# Autodesk Inventor assembly: Geeetech GT9S2 Extruder
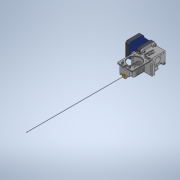
[picture p0: Inventor's stored thumbnail of the model, 180x180]
Saved by Autodesk Inventor 2020 (Build 240168000, 168)
## iProperties
Created: 2018-11-15
Part Number: Geeetech GT9S2 Extruder
Document SubType Name: Assembly
Designer: LillaHunden
Mass: 246.363 g
Surface Area: 552.129 cm^2
Volume: 126.998 cm^3
Density: 1.9399 g/cm^3
Author: LillaHunden
## Documents named in this file (24)
- C:\Users\LillaHunden\Documents\Inventor\3dprinter\3dPrinter\Geeetech GT9S2 Extruder\Geeetech GT9S2 Extruder.iam
- C:\Users\LillaHunden\Documents\Inventor\3dprinter\3dPrinter\Geeetech GT9S2 Extruder\Cooling fin.ipt
- C:\Users\LillaHunden\Documents\Inventor\3dprinter\3dPrinter\Geeetech GT9S2 Extruder\extruder body.ipt
- C:\Users\LillaHunden\Documents\Inventor\3dprinter\3dPrinter\Geeetech GT9S2 Extruder\fan bracket.ipt
- C:\Users\LillaHunden\Documents\Inventor\3dprinter\3dPrinter\Geeetech GT9S2 Extruder\feeder tube.ipt
- C:\Users\LillaHunden\Documents\Inventor\3dprinter\3dPrinter\Geeetech GT9S2 Extruder\hotend.ipt
- C:\Users\LillaHunden\Documents\Inventor\3dprinter\3dPrinter\Geeetech GT9S2 Extruder\nozzel.ipt
- C:\Users\LillaHunden\Documents\Inventor\3dprinter\3dPrinter\Geeetech GT9S2 Extruder\Geeetech GT9S2 Extruder\Design Accelerator\Bolted Connection1.iam
- C:\Users\LillaHunden\Documents\Inventor\3dprinter\3dPrinter\Geeetech GT9S2 Extruder\Geeetech GT9S2 Extruder\Design Accelerator\Bolted Connection2.iam
- C:\Users\LillaHunden\Documents\Inventor\3dprinter\3dPrinter\Geeetech GT9S2 Extruder\roller bracket.ipt
- C:\Users\LillaHunden\Documents\Inventor\3dprinter\3dPrinter\Geeetech GT9S2 Extruder\roller bearing.ipt
- C:\Users\LillaHunden\Documents\Inventor\3dprinter\3dPrinter\Geeetech GT9S2 Extruder\roller pin.ipt
- C:\Users\LillaHunden\Documents\Inventor\3dprinter\3dPrinter\Geeetech GT9S2 Extruder\roller.ipt
- C:\Users\LillaHunden\Documents\Inventor\3dprinter\3dPrinter\Nema17 import\Nema 17HS4401-S.ipt
- C:\Users\LillaHunden\Documents\Inventor\3dprinter\3dPrinter\Geeetech GT9S2 Extruder\Geeetech GT9S2 Extruder\Design Accelerator\Bolted Connection3.iam
- C:\Users\LillaHunden\Documents\Inventor\3dprinter\3dPrinter\Geeetech GT9S2 Extruder\Fillament hob.ipt
- C:\Users\LillaHunden\Documents\Inventor\3dprinter\3dPrinter\Geeetech GT9S2 Extruder\fillament guide screw.ipt
- C:\Users\LillaHunden\Documents\Inventor\3dprinter\3dPrinter\Geeetech GT9S2 Extruder\Geeetech GT9S2 Extruder\Design Accelerator\Bolted Connection4.iam
- C:\Users\LillaHunden\Documents\Inventor\3dprinter\3dPrinter\dummyAxis.ipt
- C:\Users\LillaHunden\Documents\Inventor\Content Center Files\R2020\en-US\DIN 912\DIN 912 - M3 x 0,5 x 8 x 6,75.ipt
- C:\Users\LillaHunden\Documents\Inventor\Content Center Files\R2020\en-US\DIN 912\DIN 912 - M2,5 x 0,45 x 5 x 3,875.ipt
- C:\Users\LillaHunden\Documents\Inventor\Content Center Files\R2020\en-US\DIN 912\DIN 912 - M3 x 0,5 x 30 x 18.ipt
- C:\Users\LillaHunden\Documents\Inventor\Content Center Files\R2020\en-US\DIN 912\DIN 912 - M3 x 0,5 x 5 x 3,75.ipt
- C:\Users\LillaHunden\Documents\Inventor\Content Center Files\R2020\en-US\AS 1421(1)\AS 1421 - M4x12 Cone Point.ipt
## Components (27 placed, 20 different names)
1. Cooling fin:1 — Mate:5, Mate:6
2. extruder body:1 — Mate:1, Mate:2, Mate:9, Mate:17, Angle:3, Mate:18, Insert:1, Mate:22, Mate:23, Insert:2, Insert:3, Insert:4, Mate:33, Mate:36
3. fan bracket:1 — Mate:9, Angle:1, Angle:2, Flush:1, Insert:5, Insert:6, Mate:29, Mate:31, Mate:35
4. feeder tube:1 — Mate:1, Mate:2, Mate:3, Mate:4, Mate:5, Mate:6
5. hotend:1 — Mate:7, Mate:8, Angle:1, Angle:2, Flush:1, Mate:30, Mate:32
6. nozzel:1 — Mate:3, Mate:4, Mate:7, Mate:8, Flush:3
7. Bolted Connection:1 [sub-assembly] — Mate:29, Mate:30
8. Bolted Connection:2 [sub-assembly] — Mate:31, Mate:32
9. roller bracket:1 — Mate:16, Insert:1, Insert:7
10. roller bearing:1 — Mate:14, Flush:2, Mate:15
11. roller pin:1 — Mate:15, Mate:16
12. roller:1 — Mate:14, Flush:2
13. Nema 17HS4401-S:1 — Mate:17, Angle:3, Mate:18, Angle:4, Angle:5, Tangent:1, Mate:21, Mate:34
14. Bolted Connection:3 [sub-assembly] — Mate:33, Mate:34
15. Fillament hob:1 — Angle:4, Angle:5, Tangent:1, Mate:21
16. fillament guide screw:1 — Mate:22, Mate:23
17. AS 1421 Cone Point - Metric M4x12 Cone Point:1
18. AS 1421 Cone Point - Metric M4x12 Cone Point:2
19. DIN 912 - replaced by DIN EN ISO 4762 M3 x 5:3 — Insert:2
20. DIN 912 - replaced by DIN EN ISO 4762 M3 x 5:4 — Insert:3
21. DIN 912 - replaced by DIN EN ISO 4762 M3 x 30:1 — Insert:4
22. Bolted Connection:4 [sub-assembly] — Mate:35, Mate:36
23. DIN 912 - replaced by DIN EN ISO 4762 M2,5 x 5:1
24. DIN 912 - replaced by DIN EN ISO 4762 M3 x 8:4 — Insert:5
25. DIN 912 - replaced by DIN EN ISO 4762 M3 x 8:5 — Insert:6
26. DIN 912 - replaced by DIN EN ISO 4762 M3 x 8:6 — Insert:7
27. dummyAxis:1 — Flush:3
## Relationships (44: Mate 28, Insert 7, Angle 5, Flush 3, Tangent 1)
- Mate:1: extruder body:1 ↔ feeder tube:1
- Mate:2 (1.35 mm): extruder body:1 ↔ feeder tube:1
- Mate:3: feeder tube:1 ↔ nozzel:1
- Mate:4 (0.3 mm): feeder tube:1 ↔ nozzel:1
- Mate:5: Cooling fin:1 ↔ feeder tube:1
- Mate:6 (4 mm): Cooling fin:1 ↔ feeder tube:1
- Mate:7: hotend:1 ↔ nozzel:1
- Mate:8: hotend:1 ↔ nozzel:1
- Mate:9: extruder body:1 ↔ fan bracket:1
- Angle:1 (0 deg): fan bracket:1 ↔ hotend:1
- Angle:2 (180 deg): fan bracket:1 ↔ hotend:1
- Flush:1: fan bracket:1 ↔ hotend:1
- Mate:14: roller bearing:1 ↔ roller:1
- Flush:2 (-0.5 mm): roller bearing:1 ↔ roller:1
- Mate:15: roller bearing:1 ↔ roller pin:1
- Mate:16: roller bracket:1 ↔ roller pin:1
- Mate:17: extruder body:1 ↔ Nema 17HS4401-S:1
- Angle:3 (0 deg): extruder body:1 ↔ Nema 17HS4401-S:1
- Mate:18: extruder body:1 ↔ Nema 17HS4401-S:1
- Insert:1: extruder body:1 ↔ roller bracket:1
- Angle:4 (180 deg): Nema 17HS4401-S:1 ↔ Fillament hob:1
- Angle:5 (180 deg): Nema 17HS4401-S:1 ↔ Fillament hob:1
- Tangent:1: Nema 17HS4401-S:1 ↔ Fillament hob:1
- Mate:21 (6 mm): Nema 17HS4401-S:1 ↔ Fillament hob:1
- Mate:22: extruder body:1 ↔ fillament guide screw:1
- Mate:23: extruder body:1 ↔ fillament guide screw:1
- [Mate]: roller bracket:1 ↔ AS 1421 Cone Point - Metric M4x12 Cone Point:1
- [Mate]: roller bracket:1 ↔ AS 1421 Cone Point - Metric M4x12 Cone Point:2
- Insert:2: extruder body:1 ↔ DIN 912 - replaced by DIN EN ISO 4762 M3 x 5:3
- Insert:3: extruder body:1 ↔ DIN 912 - replaced by DIN EN ISO 4762 M3 x 5:4
- Insert:4: extruder body:1 ↔ DIN 912 - replaced by DIN EN ISO 4762 M3 x 30:1
- [Mate]: hotend:1 ↔ DIN 912 - replaced by DIN EN ISO 4762 M2,5 x 5:1
- Insert:5: fan bracket:1 ↔ DIN 912 - replaced by DIN EN ISO 4762 M3 x 8:4
- Insert:6: fan bracket:1 ↔ DIN 912 - replaced by DIN EN ISO 4762 M3 x 8:5
- Insert:7: roller bracket:1 ↔ DIN 912 - replaced by DIN EN ISO 4762 M3 x 8:6
- Flush:3: nozzel:1 ↔ dummyAxis:1
- Mate:29: fan bracket:1 ↔ Bolted Connection:1
- Mate:30: hotend:1 ↔ Bolted Connection:1
- Mate:31: fan bracket:1 ↔ Bolted Connection:2
- Mate:32: hotend:1 ↔ Bolted Connection:2
- Mate:33: extruder body:1 ↔ Bolted Connection:3
- Mate:34: Nema 17HS4401-S:1 ↔ Bolted Connection:3
- Mate:35: fan bracket:1 ↔ Bolted Connection:4
- Mate:36: extruder body:1 ↔ Bolted Connection:4
